# Autodesk Inventor assembly: Protocube
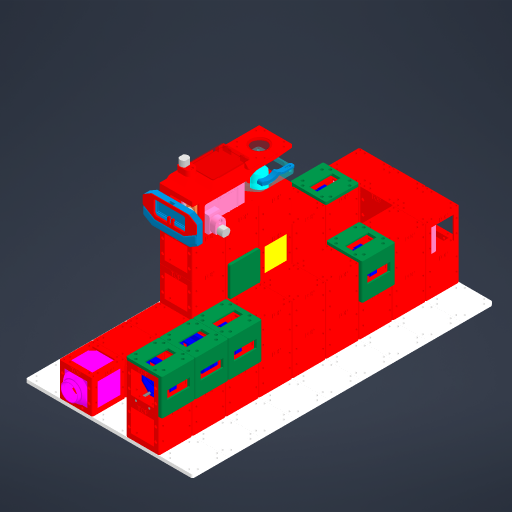
[picture p0: Inventor's stored thumbnail of the model, 512x512]
Saved by Autodesk Inventor 2023.4 (Build 274418000, 418)
## iProperties
Created: 2022-08-13
Part Number: Protocube
Document SubType Name: Assembly
Designer: xSibe
Author: xSibe
## Documents named in this file (17)
- C:\.Laptop\.Work\Projects\Project Protocube\Protocube\CAD, STL, OBJ Files\1 CAD\Protocube.iam
- C:\.Laptop\.Work\Projects\Project Protocube\Protocube\CAD, STL, OBJ Files\1 CAD\Baseplates\Baseplate 9x5 V5.ipt
- C:\.Laptop\.Work\Projects\Project Protocube\Protocube\CAD, STL, OBJ Files\1 CAD\Lens\Cube 1x1 V5 (Half Inch Lens).iam
- C:\.Laptop\.Work\Projects\Project Protocube\Protocube\CAD, STL, OBJ Files\1 CAD\Mirror\Cube 1x1 V5 (Mirror Horizontal).iam
- C:\.Laptop\.Work\Projects\Project Protocube\Protocube\CAD, STL, OBJ Files\1 CAD\Cubes\Cube 1x1 V5 Closed Horizontal.iam
- C:\.Laptop\.Work\Projects\Project Protocube\Protocube\CAD, STL, OBJ Files\1 CAD\Lens\Cube 1x1 V5 (One Inch Lens).iam
- C:\.Laptop\.Work\Projects\Project Protocube\Protocube\CAD, STL, OBJ Files\1 CAD\XYZ Stage\XYZ Stage V5.iam
- C:\.Laptop\.Work\Projects\Project Protocube\Protocube\CAD, STL, OBJ Files\1 CAD\Mirror\Cube 1x1 V5 (Mirror Vertical).iam
- C:\.Laptop\.Work\Projects\Project Protocube\Protocube\CAD, STL, OBJ Files\1 CAD\Laser\Cube 1x1 V5 (USB Laser).iam
- C:\.Laptop\.Work\Projects\Project Protocube\Protocube\CAD, STL, OBJ Files\1 CAD\Camera\Cube 1x1 V5 (Camera).iam
- C:\.Laptop\.Work\Projects\Project Protocube\Protocube\CAD, STL, OBJ Files\1 CAD\Dichroic\Cube 1x1 V5 (Dichroic).iam
- C:\.Laptop\.Work\Projects\Project Protocube\Protocube\CAD, STL, OBJ Files\1 CAD\Objective\Cube 1x1 V5 (Objective).iam
- C:\.Laptop\.Work\Projects\Project Protocube\Protocube\CAD, STL, OBJ Files\1 CAD\Gamepad\Gamepad Enclosure.iam
- C:\.Laptop\.Work\Projects\Project Protocube\Protocube\CAD, STL, OBJ Files\1 CAD\Sample\Cube (Sample).iam
- C:\.Laptop\.Work\Projects\Project Protocube\Protocube\CAD, STL, OBJ Files\1 CAD\Cubes\Cube 1x1 V5.iam
- C:\.Laptop\.Work\Projects\Project Protocube\Protocube\CAD, STL, OBJ Files\1 CAD\Covers\Outer Cover Side.ipt
- C:\.Laptop\.Work\Projects\Project Protocube\Protocube\CAD, STL, OBJ Files\1 CAD\Lens\Cube 1x1 V5 (SM1 Lens).iam
## Components (44 placed, 16 different names)
1. Baseplate 9x5 V5:1 — Mate:60, Mate:61, Mate:62, Mate:65, Mate:66, Mate:67, Mate:69, Mate:70, Mate:71, Mate:93, Mate:94, Mate:95, Mate:101, Mate:102, Mate:103, Mate:107, Mate:108, Mate:109, Mate:118, Mate:119, Mate:120, Mate:121, Mate:122, Mate:123, Mate:136, Mate:137, Mate:138
2. Outer Cover Side:1 — Mate:130, Mate:131, Mate:132
3. Outer Cover Side:2 — Mate:133, Mate:134, Mate:135
4. Cube 1x1 V5 (Mirror Horizontal):1 [sub-assembly] — Mate:81, Flush:14, Flush:15
5. Cube 1x1 V5 (Mirror Horizontal):2 [sub-assembly] — Flush:16, Flush:17, Mate:82
6. Cube 1x1 V5 (One Inch Lens):3 [sub-assembly] — Mate:121, Mate:122, Mate:123, Mate:124, Mate:125, Mate:126
7. Cube 1x1 V5 (Half Inch Lens):1 [sub-assembly] — Mate:77, Flush:8, Flush:9
8. Cube 1x1 V5 (One Inch Lens):1 [sub-assembly] — Mate:96, Flush:87, Flush:88
9. Cube 1x1 V5 (One Inch Lens):2 [sub-assembly] — Mate:97, Flush:89, Flush:90
10. Cube 1x1 V5 (Mirror Vertical):1 [sub-assembly] — Mate:101, Mate:102, Mate:103, Mate:110, Flush:91, Flush:92
11. Cube 1x1 V5 (USB Laser):1 [sub-assembly] — Mate:104, Mate:105, Mate:106
12. Cube 1x1 V5 (Camera):1 [sub-assembly] — Mate:107, Mate:108, Mate:109
13. Cube 1x1 V5 (Dichroic):1 [sub-assembly] — Mate:110, Flush:91, Flush:92, Mate:111, Flush:93, Flush:94
14. Cube 1x1 V5 (Objective):1 [sub-assembly] — Mate:111, Flush:93, Flush:94, Mate:113, Mate:114, Mate:115
15. Gamepad Enclosure:1 [sub-assembly] — Mate:112, Mate:116, Mate:117
16. Cube (Sample):1 [sub-assembly] — Mate:118, Mate:119, Mate:120
17. XYZ Stage V5:1 [sub-assembly] — Mate:112, Mate:113, Mate:114, Mate:115, Mate:116, Mate:117
18. Cube 1x1 V5 (SM1 Lens):1 [sub-assembly] — Mate:136, Mate:137, Mate:138
19. Cube 1x1 V5:1 [sub-assembly] — Mate:124, Mate:125, Mate:126, Mate:127, Mate:128, Mate:129, Mate:130, Mate:131, Mate:132, Mate:133, Mate:134, Mate:135
20. Cube 1x1 V5 Closed Horizontal:13 [sub-assembly] — Flush:3, Mate:80, Flush:13
21. Cube 1x1 V5 Closed Horizontal:17 [sub-assembly] — Flush:20, Flush:21, Mate:84
22. Cube 1x1 V5 Closed Horizontal:27 [sub-assembly] — Mate:127, Mate:128, Mate:129
23. Cube 1x1 V5 Closed Horizontal:1 [sub-assembly] — Mate:60, Mate:61, Mate:62, Mate:104, Mate:105, Mate:106
24. Cube 1x1 V5 Closed Horizontal:2 [sub-assembly]
25. Cube 1x1 V5 Closed Horizontal:3 [sub-assembly] — Mate:77, Flush:8, Flush:9
26. Cube 1x1 V5 Closed Horizontal:4 [sub-assembly] — Flush:2, Mate:78, Flush:10
27. Cube 1x1 V5 Closed Horizontal:5 [sub-assembly]
28. Cube 1x1 V5 Closed Horizontal:6 [sub-assembly]
29. Cube 1x1 V5 Closed Horizontal:7 [sub-assembly] — Mate:96, Flush:87, Flush:88
30. Cube 1x1 V5 Closed Horizontal:8 [sub-assembly] — Flush:3, Mate:80, Flush:13
31. Cube 1x1 V5 Closed Horizontal:9 [sub-assembly] — Mate:81, Flush:14, Flush:15
32. Cube 1x1 V5 Closed Horizontal:10 [sub-assembly] — Flush:2, Mate:78, Flush:10
33. Cube 1x1 V5 Closed Horizontal:11 [sub-assembly]
34. Cube 1x1 V5 Closed Horizontal:12 [sub-assembly]
35. Cube 1x1 V5 Closed Horizontal:14 [sub-assembly] — Mate:65, Mate:66, Mate:67, Flush:16, Flush:17, Mate:82
36. Cube 1x1 V5 Closed Horizontal:15 [sub-assembly] — Mate:97, Flush:89, Flush:90
37. Cube 1x1 V5 Closed Horizontal:16 [sub-assembly] — Flush:20, Mate:84, Flush:21
38. Cube 1x1 V5 Closed Horizontal:18 [sub-assembly] — Mate:69, Mate:70, Mate:71, Flush:5, Mate:91, Flush:27
39. Cube 1x1 V5 Closed Horizontal:19 [sub-assembly]
40. Cube 1x1 V5 Closed Horizontal:20 [sub-assembly]
41. Cube 1x1 V5 Closed Horizontal:21 [sub-assembly] — Flush:5, Mate:91, Flush:27
42. Cube 1x1 V5 Closed Horizontal:22 [sub-assembly]
43. Cube 1x1 V5 Closed Horizontal:25 [sub-assembly] — Mate:93, Mate:94, Mate:95
44. Cube 1x1 V5 Closed Horizontal:26 [sub-assembly]
## Component patterns: (9 elements, first: Cube 1x1 V5 Closed Horizontal:1), (3 elements, first: Cube 1x1 V5 Closed Horizontal:10), (3 elements, first: Cube 1x1 V5 Closed Horizontal:14), (3 elements, first: Cube 1x1 V5 Closed Horizontal:18), (2 elements, first: Cube 1x1 V5 Closed Horizontal:21), (2 elements, first: Cube 1x1 V5 Closed Horizontal:25)
## Relationships (81: Mate 59, Flush 22)
- Mate:60: Baseplate 9x5 V5:1 ↔ Cube 1x1 V5 Closed Horizontal:1
- Mate:61: Baseplate 9x5 V5:1 ↔ Cube 1x1 V5 Closed Horizontal:1
- Mate:62: Baseplate 9x5 V5:1 ↔ Cube 1x1 V5 Closed Horizontal:1
- Flush:2: Cube 1x1 V5 Closed Horizontal:4 ↔ Cube 1x1 V5 Closed Horizontal:10
- Flush:3: Cube 1x1 V5 Closed Horizontal:13 ↔ Cube 1x1 V5 Closed Horizontal:8
- Mate:65: Baseplate 9x5 V5:1 ↔ Cube 1x1 V5 Closed Horizontal:14
- Mate:66: Baseplate 9x5 V5:1 ↔ Cube 1x1 V5 Closed Horizontal:14
- Mate:67: Baseplate 9x5 V5:1 ↔ Cube 1x1 V5 Closed Horizontal:14
- Mate:69: Baseplate 9x5 V5:1 ↔ Cube 1x1 V5 Closed Horizontal:18
- Mate:70: Baseplate 9x5 V5:1 ↔ Cube 1x1 V5 Closed Horizontal:18
- Mate:71: Baseplate 9x5 V5:1 ↔ Cube 1x1 V5 Closed Horizontal:18
- Flush:5: Cube 1x1 V5 Closed Horizontal:18 ↔ Cube 1x1 V5 Closed Horizontal:21
- Mate:77: Cube 1x1 V5 (Half Inch Lens):1 ↔ Cube 1x1 V5 Closed Horizontal:3
- Flush:8: Cube 1x1 V5 (Half Inch Lens):1 ↔ Cube 1x1 V5 Closed Horizontal:3
- Flush:9: Cube 1x1 V5 (Half Inch Lens):1 ↔ Cube 1x1 V5 Closed Horizontal:3
- Mate:78: Cube 1x1 V5 Closed Horizontal:4 ↔ Cube 1x1 V5 Closed Horizontal:10
- Flush:10: Cube 1x1 V5 Closed Horizontal:4 ↔ Cube 1x1 V5 Closed Horizontal:10
- Mate:80: Cube 1x1 V5 Closed Horizontal:13 ↔ Cube 1x1 V5 Closed Horizontal:8
- Flush:13: Cube 1x1 V5 Closed Horizontal:13 ↔ Cube 1x1 V5 Closed Horizontal:8
- Mate:81: Cube 1x1 V5 (Mirror Horizontal):1 ↔ Cube 1x1 V5 Closed Horizontal:9
- Flush:14: Cube 1x1 V5 (Mirror Horizontal):1 ↔ Cube 1x1 V5 Closed Horizontal:9
- Flush:15: Cube 1x1 V5 (Mirror Horizontal):1 ↔ Cube 1x1 V5 Closed Horizontal:9
- Flush:16: Cube 1x1 V5 (Mirror Horizontal):2 ↔ Cube 1x1 V5 Closed Horizontal:14
- Flush:17: Cube 1x1 V5 (Mirror Horizontal):2 ↔ Cube 1x1 V5 Closed Horizontal:14
- Mate:82: Cube 1x1 V5 (Mirror Horizontal):2 ↔ Cube 1x1 V5 Closed Horizontal:14
- Flush:20: Cube 1x1 V5 Closed Horizontal:17 ↔ Cube 1x1 V5 Closed Horizontal:16
- Flush:21: Cube 1x1 V5 Closed Horizontal:17 ↔ Cube 1x1 V5 Closed Horizontal:16
- Mate:84: Cube 1x1 V5 Closed Horizontal:17 ↔ Cube 1x1 V5 Closed Horizontal:16
- Mate:91: Cube 1x1 V5 Closed Horizontal:18 ↔ Cube 1x1 V5 Closed Horizontal:21
- Flush:27: Cube 1x1 V5 Closed Horizontal:18 ↔ Cube 1x1 V5 Closed Horizontal:21
- Mate:93: Baseplate 9x5 V5:1 ↔ Cube 1x1 V5 Closed Horizontal:25
- Mate:94: Baseplate 9x5 V5:1 ↔ Cube 1x1 V5 Closed Horizontal:25
- Mate:95: Baseplate 9x5 V5:1 ↔ Cube 1x1 V5 Closed Horizontal:25
- Mate:96: Cube 1x1 V5 (One Inch Lens):1 ↔ Cube 1x1 V5 Closed Horizontal:7
- Flush:87: Cube 1x1 V5 (One Inch Lens):1 ↔ Cube 1x1 V5 Closed Horizontal:7
- Flush:88: Cube 1x1 V5 (One Inch Lens):1 ↔ Cube 1x1 V5 Closed Horizontal:7
- Mate:97: Cube 1x1 V5 (One Inch Lens):2 ↔ Cube 1x1 V5 Closed Horizontal:15
- Flush:89: Cube 1x1 V5 (One Inch Lens):2 ↔ Cube 1x1 V5 Closed Horizontal:15
- Flush:90: Cube 1x1 V5 (One Inch Lens):2 ↔ Cube 1x1 V5 Closed Horizontal:15
- Mate:101: Baseplate 9x5 V5:1 ↔ Cube 1x1 V5 (Mirror Vertical):1
- Mate:102: Baseplate 9x5 V5:1 ↔ Cube 1x1 V5 (Mirror Vertical):1
- Mate:103: Baseplate 9x5 V5:1 ↔ Cube 1x1 V5 (Mirror Vertical):1
- Mate:104: Cube 1x1 V5 (USB Laser):1 ↔ Cube 1x1 V5 Closed Horizontal:1
- Mate:105: Cube 1x1 V5 (USB Laser):1 ↔ Cube 1x1 V5 Closed Horizontal:1
- Mate:106: Cube 1x1 V5 (USB Laser):1 ↔ Cube 1x1 V5 Closed Horizontal:1
- Mate:107: Baseplate 9x5 V5:1 ↔ Cube 1x1 V5 (Camera):1
- Mate:108: Baseplate 9x5 V5:1 ↔ Cube 1x1 V5 (Camera):1
- Mate:109: Baseplate 9x5 V5:1 ↔ Cube 1x1 V5 (Camera):1
- Mate:110: Cube 1x1 V5 (Mirror Vertical):1 ↔ Cube 1x1 V5 (Dichroic):1
- Flush:91: Cube 1x1 V5 (Mirror Vertical):1 ↔ Cube 1x1 V5 (Dichroic):1
- Flush:92: Cube 1x1 V5 (Mirror Vertical):1 ↔ Cube 1x1 V5 (Dichroic):1
- Mate:111: Cube 1x1 V5 (Dichroic):1 ↔ Cube 1x1 V5 (Objective):1
- Flush:93: Cube 1x1 V5 (Dichroic):1 ↔ Cube 1x1 V5 (Objective):1
- Flush:94: Cube 1x1 V5 (Dichroic):1 ↔ Cube 1x1 V5 (Objective):1
- Mate:112: Gamepad Enclosure:1 ↔ XYZ Stage V5:1
- Mate:113: Cube 1x1 V5 (Objective):1 ↔ XYZ Stage V5:1
- Mate:114: Cube 1x1 V5 (Objective):1 ↔ XYZ Stage V5:1
- Mate:115: Cube 1x1 V5 (Objective):1 ↔ XYZ Stage V5:1
- Mate:116: Gamepad Enclosure:1 ↔ XYZ Stage V5:1
- Mate:117: Gamepad Enclosure:1 ↔ XYZ Stage V5:1
- Mate:118: Baseplate 9x5 V5:1 ↔ Cube (Sample):1
- Mate:119: Baseplate 9x5 V5:1 ↔ Cube (Sample):1
- Mate:120: Baseplate 9x5 V5:1 ↔ Cube (Sample):1
- Mate:121: Baseplate 9x5 V5:1 ↔ Cube 1x1 V5 (One Inch Lens):3
- Mate:122: Baseplate 9x5 V5:1 ↔ Cube 1x1 V5 (One Inch Lens):3
- Mate:123: Baseplate 9x5 V5:1 ↔ Cube 1x1 V5 (One Inch Lens):3
- Mate:124: Cube 1x1 V5 (One Inch Lens):3 ↔ Cube 1x1 V5:1
- Mate:125: Cube 1x1 V5 (One Inch Lens):3 ↔ Cube 1x1 V5:1
- Mate:126: Cube 1x1 V5 (One Inch Lens):3 ↔ Cube 1x1 V5:1
- Mate:127: Cube 1x1 V5:1 ↔ Cube 1x1 V5 Closed Horizontal:27
- Mate:128: Cube 1x1 V5:1 ↔ Cube 1x1 V5 Closed Horizontal:27
- Mate:129: Cube 1x1 V5:1 ↔ Cube 1x1 V5 Closed Horizontal:27
- Mate:130: Outer Cover Side:1 ↔ Cube 1x1 V5:1
- Mate:131: Outer Cover Side:1 ↔ Cube 1x1 V5:1
- Mate:132: Outer Cover Side:1 ↔ Cube 1x1 V5:1
- Mate:133: Outer Cover Side:2 ↔ Cube 1x1 V5:1
- Mate:134: Outer Cover Side:2 ↔ Cube 1x1 V5:1
- Mate:135: Outer Cover Side:2 ↔ Cube 1x1 V5:1
- Mate:136: Baseplate 9x5 V5:1 ↔ Cube 1x1 V5 (SM1 Lens):1
- Mate:137: Baseplate 9x5 V5:1 ↔ Cube 1x1 V5 (SM1 Lens):1
- Mate:138: Baseplate 9x5 V5:1 ↔ Cube 1x1 V5 (SM1 Lens):1
